# Autodesk Inventor assembly: curve+flat
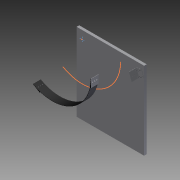
[picture p0: Inventor's stored thumbnail of the model, 180x180]
Saved by Autodesk Inventor 2011 SP1 (Build 150282100, 282)
## iProperties
Created: 2013-01-18
Part Number: curve+flat
Document SubType Name: Assembly
Designer: wes
Author: wes
## Documents named in this file (6)
- F:\ALL FILES\My Documents\GitHub\2013CAD\2013 robot\CurvedShooter\curve+flat.iam
- F:\ALL FILES\My Documents\GitHub\2013CAD\2013 robot\CurvedShooter\ajustableBase w mounting holes.ipt
- F:\ALL FILES\My Documents\GitHub\2013CAD\2013 robot\CurvedShooter\curveBracket.ipt
- F:\ALL FILES\My Documents\GitHub\2013CAD\2013 robot\CurvedShooter\Common Chassis Parts\.25 diameter 2'' bolt.ipt
- F:\ALL FILES\My Documents\GitHub\2013CAD\2013 robot\CurvedShooter\120 degree curved track.ipt
- F:\ALL FILES\My Documents\GitHub\2013CAD\2013 robot\CurvedShooter\Common Chassis Parts\.25 diameter 1'' bolt.ipt
## Components (10 placed, 5 different names)
1. ajustableBase w mounting holes:1 — Insert:14, Insert:15, Insert:16, Insert:17, Insert:18, Insert:19
2. curveBracket:1 — Insert:18, Insert:19
3. .25 diameter 2'' bolt:1 — Insert:14
4. .25 diameter 2'' bolt:2 — Insert:15
5. .25 diameter 2'' bolt:3 — Insert:17
6. .25 diameter 2'' bolt:4 — Insert:16
7. 120 degree curved track:1 — Insert:11, Insert:12, Insert:13
8. .25 diameter 1'' bolt:1 — Insert:12
9. .25 diameter 1'' bolt:2 — Insert:13
10. .25 diameter 1'' bolt:3 — Insert:11
## Relationships (9: Insert 9)
- Insert:11: 120 degree curved track:1 ↔ .25 diameter 1'' bolt:3
- Insert:12: 120 degree curved track:1 ↔ .25 diameter 1'' bolt:1
- Insert:13: 120 degree curved track:1 ↔ .25 diameter 1'' bolt:2
- Insert:14: ajustableBase w mounting holes:1 ↔ .25 diameter 2'' bolt:1
- Insert:15: ajustableBase w mounting holes:1 ↔ .25 diameter 2'' bolt:2
- Insert:16: ajustableBase w mounting holes:1 ↔ .25 diameter 2'' bolt:4
- Insert:17: ajustableBase w mounting holes:1 ↔ .25 diameter 2'' bolt:3
- Insert:18: ajustableBase w mounting holes:1 ↔ curveBracket:1
- Insert:19: ajustableBase w mounting holes:1 ↔ curveBracket:1
